# Autodesk Inventor assembly: matrix
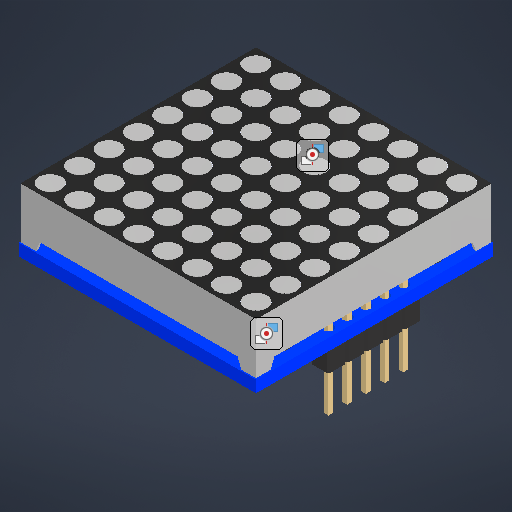
[picture p0: Inventor's stored thumbnail of the model, 512x512]
Saved by Autodesk Inventor 2025.2 (Build 292293000, 293)
## iProperties
Created: 2025-06-28
Part Number: matrix
Document SubType Name: Assembly
Designer: micyg
Author: micyg
## Documents named in this file (5)
- D:\Projects\VirtualPets\VirtualBlob\Mechanical\matrix\matrix.iam
- D:\Projects\VirtualPets\VirtualBlob\Mechanical\matrix\1088AS.ipt
- D:\Projects\VirtualPets\VirtualBlob\Mechanical\matrix\MAX7219.ipt
- D:\Projects\VirtualPets\VirtualBlob\Mechanical\matrix\PCB.ipt
- D:\Projects\VirtualPets\VirtualBlob\Mechanical\matrix\PinHeader_1x05_P2.54mm_Vertical.ipt
## Components (5 placed, 4 different names)
1. 1088AS:1 — Mate:20, Mate:21, Mate:22
2. MAX7219:1 — Flush:1, Mate:8, Mate:13
3. PCB:1 — Flush:1, Mate:8, Mate:13, Mate:14, Mate:15, Mate:16, Mate:17, Mate:18, Angle:1, Mate:19, Angle:2, Mate:20, Mate:21, Mate:22
4. PinHeader_1x05_P2.54mm_Vertical:1 — Mate:15, Mate:16, Mate:17, Angle:1
5. PinHeader_1x05_P2.54mm_Vertical:2 — Mate:14, Mate:18, Mate:19, Angle:2
## Relationships (14: Mate 11, Angle 2, Flush 1)
- Flush:1 (-8 mm): MAX7219:1 ↔ PCB:1
- Mate:8 (-19 mm): MAX7219:1 ↔ PCB:1
- Mate:13: MAX7219:1 ↔ PCB:1
- Mate:14: PCB:1 ↔ PinHeader_1x05_P2.54mm_Vertical:2
- Mate:15: PCB:1 ↔ PinHeader_1x05_P2.54mm_Vertical:1
- Mate:16 (-0.32 mm): PCB:1 ↔ PinHeader_1x05_P2.54mm_Vertical:1
- Mate:17 (-0.32 mm): PCB:1 ↔ PinHeader_1x05_P2.54mm_Vertical:1
- Mate:18 (-0.32 mm): PCB:1 ↔ PinHeader_1x05_P2.54mm_Vertical:2
- Angle:1 (0 deg): PCB:1 ↔ PinHeader_1x05_P2.54mm_Vertical:1
- Mate:19 (-0.32 mm): PCB:1 ↔ PinHeader_1x05_P2.54mm_Vertical:2
- Angle:2 (0 deg): PCB:1 ↔ PinHeader_1x05_P2.54mm_Vertical:2
- Mate:20: 1088AS:1 ↔ PCB:1
- Mate:21: 1088AS:1 ↔ PCB:1
- Mate:22: 1088AS:1 ↔ PCB:1
